# Autodesk Inventor assembly: 24T HS Gear Cut
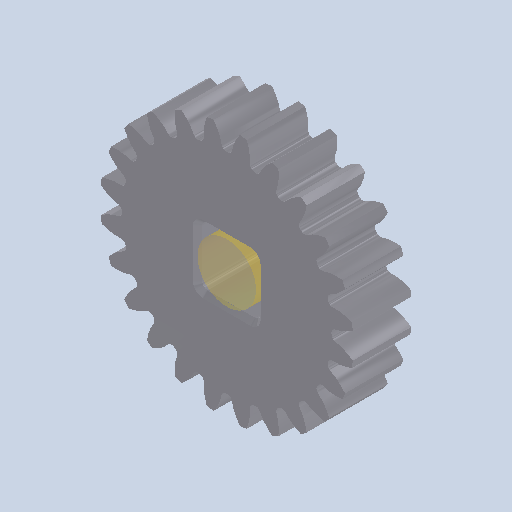
[picture p0: Inventor's stored thumbnail of the model, 512x512]
Saved by Autodesk Inventor 2025.2 (Build 292293000, 293)
## iProperties
Created: 2025-03-23
Part Number: 24T HS Gear Cut
Document SubType Name: Assembly
Designer: roejo
Author: roejo
## Documents named in this file (3)
- C:\1629X-7700R-Worlds-Bot\VEX-CAD-Inventor-1.4.2\Motion\Gears\HS Gear\24T HS Gear Cut.iam
- C:\1629X-7700R-Worlds-Bot\VEX-CAD-Inventor-1.4.2\Motion\Gears\HS Gear\HS 24T Gear, No Insert.iam
- C:\1629X-7700R-Worlds-Bot\VEX-CAD-Inventor-1.4.2\Motion\Gears\HS Gear.iam
## Components (1 placed, 1 different names)
1. HS 24T Gear, No Insert:1 [sub-assembly] — Mate:1
## Relationships (1: Mate 1)
- Mate:1: HS 24T Gear, No Insert:1
